# Autodesk Inventor assembly: 39197
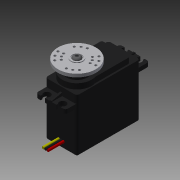
[picture p0: Inventor's stored thumbnail of the model, 180x180]
Saved by Autodesk Inventor 2018 (Build 220112000, 112)
## iProperties
Category: Servo
Company: Autodesk Inc.
Created: 2017-01-02
Part Number: 39197
Document SubType Name: Assembly
Designer: Autodesk Inc.
Vendor: Tetrix
Catalog Web Link: http://www.tetrixrobotics.com/180_Standard-Scale_HS-485HB_Servo_Motor?SKU=W39197&tp=1
Author: Autodesk Inc.
## Documents named in this file (5)
- D:\FTC 2018\FTC 2018 KOP Inventor\Tetrix\Tetrix_39197.iam
- D:\FTC 2018\FTC 2018 KOP Inventor\Tetrix\Tetrix_39197_Servo.ipt
- D:\FTC 2018\FTC 2018 KOP Inventor\Tetrix\Tetrix_39197_Metal_Horn.ipt
- D:\FTC 2018\FTC 2018 KOP Inventor\Tetrix\Tetrix_39197_Screw.ipt
- D:\FTC 2018\FTC 2018 KOP Inventor\Tetrix\Tetrix_39197_Plastic_Horn.ipt
## Components (5 placed, 5 different names)
1. Tetrix_739197_Servo — Insert:1, Insert:2
2. Tetrix_739197_Metal_Horn — Insert:2, Insert:3
3. Tetrix_739197_Screw — Insert:3
4. Tetrix_739197_Plastic_Horn — Insert:1, Insert:4
5. Tetrix_39197_Screw:2 — Insert:4
## Relationships (4: Insert 4)
- Insert:1: Tetrix_739197_Servo ↔ Tetrix_739197_Plastic_Horn
- Insert:2: Tetrix_739197_Servo ↔ Tetrix_739197_Metal_Horn
- Insert:3: Tetrix_739197_Metal_Horn ↔ Tetrix_739197_Screw
- Insert:4: Tetrix_739197_Plastic_Horn ↔ Tetrix_39197_Screw:2
